# Autodesk Inventor assembly: assembled standoffs
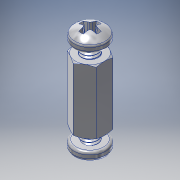
[picture p0: Inventor's stored thumbnail of the model, 180x180]
Saved by Autodesk Inventor 2016 (Build 200138000, 138)
## iProperties
Created: 2016-08-09
Part Number: assembled standoffs
Document SubType Name: Assembly
Designer: Jonathan
Author: Jonathan
## Documents named in this file (3)
- C:\Users\Jonathan\Documents\Projects\mppcInterface\4-channel\mppcInterface\cad\hardware\assembled standoffs.iam
- C:\Users\Jonathan\Documents\Projects\mppcInterface\4-channel\mppcInterface\cad\hardware\M2.5x10mm female female standoff.ipt
- C:\Users\Jonathan\Documents\Projects\mppcInterface\4-channel\mppcInterface\cad\hardware\M2.5 6mm screw.ipt
## Components (3 placed, 2 different names)
1. M2.5x10mm female female standoff:1 — Mate:1, Mate:2, Mate:3, Mate:4, Mate:6
2. M2.5 6mm screw:1 — Mate:1, Mate:2, Mate:5, Mate:6
3. M2.5 6mm screw:2 — Mate:3, Mate:4, Mate:5
## Relationships (6: Mate 6)
- Mate:1 (1.6 mm): M2.5x10mm female female standoff:1 ↔ M2.5 6mm screw:1
- Mate:2: M2.5x10mm female female standoff:1 ↔ M2.5 6mm screw:1
- Mate:3 (1.6 mm): M2.5x10mm female female standoff:1 ↔ M2.5 6mm screw:2
- Mate:4: M2.5x10mm female female standoff:1 ↔ M2.5 6mm screw:2
- Mate:5: M2.5 6mm screw:1 ↔ M2.5 6mm screw:2
- Mate:6: M2.5x10mm female female standoff:1 ↔ M2.5 6mm screw:1
